# Autodesk Inventor assembly: NewBeltGear
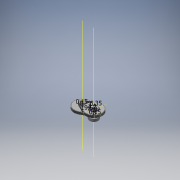
[picture p0: Inventor's stored thumbnail of the model, 180x180]
Saved by Autodesk Inventor 2018.3 (Build 223284000, 284)
## iProperties
Created: 2018-08-27
Part Number: NewBeltGear
Material: Generisch
Document SubType Name: Assembly
Designer: JochenAlt
Author: JochenAlt
## Documents named in this file (8)
- D:\Projects\Ondine\CAD\Beltdrive\Construction\NewBeltGear.iam
- D:\Projects\Ondine\CAD\Beltdrive\Construction\Input.ipt
- D:\Projects\Ondine\CAD\Beltdrive\Construction\Output.ipt
- D:\Projects\Ondine\CAD\Beltdrive\Construction\BeltGear.ipt
- D:\Projects\Ondine\CAD\Beltdrive\Construction\Zahnriemen4.ipt
- D:\Projects\Ondine\CAD\Mounting Hub.ipt
- D:\Projects\Ondine\CAD\AST_Bearings_SMR74.ipt
- C:\Users\JochenAlt\Documents\Inventor\Content Center Files\R2018\de-DE\DIN 912\DIN 912 - M3 x 0,5 x 6 x 4,75.ipt
## Components (13 placed, 7 different names)
1. Input:1 — Passend:1, Passend:2, Passend:3, Passend:13, Passend:16, Passend:17, Passend:18, Passend:19, Passend:20
2. output:1 — Passend:8, Passend:15, Einfügen:1, Einfügen:2, Einfügen:3, Einfügen:4, Passend:20
3. beltGeaR:1 — Passend:9, Passend:10, Fluchtend:1, Passend:11
4. Zahnriemen:1 — Passend:5, Passend:6, Passend:7, Passend:8, Passend:11, Passend:12, Passend:14
5. Zahnriemen:2 — Passend:2, Passend:3, Passend:4, Passend:7, Passend:10, Fluchtend:1
6. Mounting Hub:1 — Passend:12, Passend:13
7. Mounting Hub:2 — Passend:14, Passend:15
8. DIN 912 - ersetzt durch DIN EN ISO 4762 M3 x 6:1 — Einfügen:1
9. DIN 912 - ersetzt durch DIN EN ISO 4762 M3 x 6:2 — Einfügen:2
10. DIN 912 - ersetzt durch DIN EN ISO 4762 M3 x 6:3 — Einfügen:3
11. DIN 912 - ersetzt durch DIN EN ISO 4762 M3 x 6:4 — Einfügen:4
12. AST_Bearings_SMR74:1 — Passend:16, Passend:19
13. AST_Bearings_SMR74:2 — Passend:17, Passend:18
## Relationships (25: Mate 20, Insert 4, Flush 1)
- Passend:1 [Mate]: Input:1
- Passend:2 [Mate]: Input:1 ↔ Zahnriemen:2
- Passend:3 [Mate] (0.5 mm): Input:1 ↔ Zahnriemen:2
- Passend:4 [Mate]: Zahnriemen:2
- Passend:5 [Mate]: Zahnriemen:1
- Passend:6 [Mate]: Zahnriemen:1
- Passend:7 [Mate]: Zahnriemen:1 ↔ Zahnriemen:2
- Passend:8 [Mate]: output:1 ↔ Zahnriemen:1
- Passend:9 [Mate]: beltGeaR:1
- Passend:10 [Mate] (31.3 mm): beltGeaR:1 ↔ Zahnriemen:2
- Fluchtend:1 [Flush] (0.5 mm): beltGeaR:1 ↔ Zahnriemen:2
- Passend:11 [Mate] (0.5 mm): beltGeaR:1 ↔ Zahnriemen:1
- Passend:12 [Mate]: Zahnriemen:1 ↔ Mounting Hub:1
- Passend:13 [Mate]: Input:1 ↔ Mounting Hub:1
- Passend:14 [Mate]: Zahnriemen:1 ↔ Mounting Hub:2
- Passend:15 [Mate]: output:1 ↔ Mounting Hub:2
- Einfügen:1 [Insert]: output:1 ↔ DIN 912 - ersetzt durch DIN EN ISO 4762 M3 x 6:1
- Einfügen:2 [Insert]: output:1 ↔ DIN 912 - ersetzt durch DIN EN ISO 4762 M3 x 6:2
- Einfügen:3 [Insert]: output:1 ↔ DIN 912 - ersetzt durch DIN EN ISO 4762 M3 x 6:3
- Einfügen:4 [Insert]: output:1 ↔ DIN 912 - ersetzt durch DIN EN ISO 4762 M3 x 6:4
- Passend:16 [Mate]: Input:1 ↔ AST_Bearings_SMR74:1
- Passend:17 [Mate]: Input:1 ↔ AST_Bearings_SMR74:2
- Passend:18 [Mate]: Input:1 ↔ AST_Bearings_SMR74:2
- Passend:19 [Mate]: Input:1 ↔ AST_Bearings_SMR74:1
- Passend:20 [Mate] (0.2 mm): Input:1 ↔ output:1
